# Autodesk Inventor assembly: Сборка1
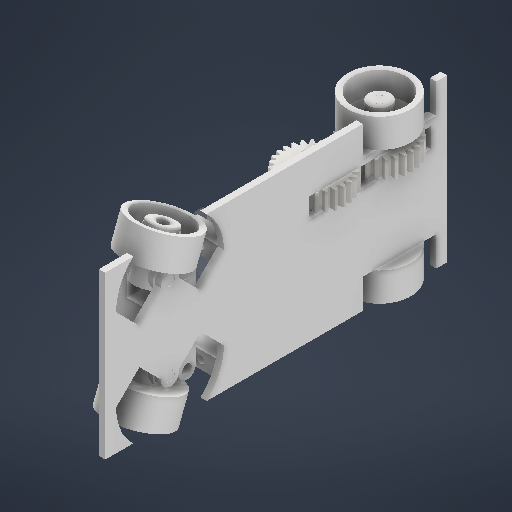
[picture p0: Inventor's stored thumbnail of the model, 512x512]
Saved by Autodesk Inventor 2026.2 (Build 302298000, 298)
## iProperties
Created: 2026-02-19
Part Number: Сборка1
Document SubType Name: Assembly
Designer: Leonid
Author: Leonid
## Documents named in this file (14)
- D:\Documents\Проекты\AutoBus\3Д модель\Сборка3.iam
- D:\Documents\Проекты\AutoBus\3Д модель\Малый сервопривод.ipt
- D:\Documents\Проекты\AutoBus\3Д модель\Рулевой толкатель на сервопривод.ipt
- D:\Documents\Проекты\AutoBus\3Д модель\Колесо переднее.ipt
- D:\Documents\Проекты\AutoBus\3Д модель\Кулак левый.ipt
- D:\Documents\Проекты\AutoBus\3Д модель\Штырь левый.ipt
- D:\Documents\Проекты\AutoBus\3Д модель\Тяга.ipt
- D:\Documents\Проекты\AutoBus\3Д модель\Кулак правый.ipt
- D:\Documents\Проекты\AutoBus\3Д модель\Штырь правый.ipt
- D:\Documents\Проекты\AutoBus\3Д модель\Вал.ipt
- D:\Documents\Проекты\AutoBus\3Д модель\Колесо заднее.ipt
- D:\Documents\Проекты\AutoBus\3Д модель\Рама3.ipt
- D:\Documents\Проекты\AutoBus\3Д модель\Мотор 15x12x10 с редуктоом.ipt
- D:\Documents\Проекты\AutoBus\3Д модель\Сборка3\Мастер проектирования\Цилиндрическое зубчатое зацепление4.iam
## Components (15 placed, 13 different names)
1. Рама3:1 — Цилиндрический:3, Совмещение:2, Заподлицо:2, Совмещение:12, Цилиндрический:16, Угол:1, Совмещение:13, Угол:2, Совмещение:19, Совмещение:20, Совмещение:24, Совмещение:25, Совмещение:26, Совмещение:28, Цилиндрический:26
2. Малый сервопривод:1 — Цилиндрический:11, Заподлицо:3, Совмещение:25, Совмещение:26
3. Кулак правый:1 — Цилиндрический:14, Совмещение:11, Совмещение:12, Цилиндрический:16, Цилиндрический:18, Заподлицо:7
4. Кулак левый:2 — Цилиндрический:3, Совмещение:2, Цилиндрический:4, Совмещение:4, Цилиндрический:13, Заподлицо:6
5. Тяга:1 — Цилиндрический:13, Цилиндрический:14, Совмещение:13, Касательность:1
6. Штырь правый:1 — Цилиндрический:17, Цилиндрический:18, Совмещение:14, Заподлицо:7
7. Штырь левый:2 — Цилиндрический:4, Цилиндрический:5, Совмещение:3, Заподлицо:6
8. Колесо переднее:1 — Совмещение:11, Цилиндрический:17, Совмещение:14
9. Колесо переднее:2 — Цилиндрический:5, Совмещение:3, Совмещение:4
10. Рулевой толкатель на сервопривод:1 — Цилиндрический:11, Заподлицо:3, Заподлицо:2, Угол:1, Угол:2, Касательность:1
11. Вал:1 — Цилиндрический:22, Заподлицо:8, Цилиндрический:23, Совмещение:27, Цилиндрический:25, Цилиндрический:26
12. Колесо заднее:1 — Цилиндрический:22, Совмещение:19, Заподлицо:8
13. Колесо заднее:2 — Цилиндрический:23, Совмещение:20
14. Мотор 15x12x10 с редуктоом:1 — Совмещение:24, Совмещение:27, Цилиндрический:24, Совмещение:29
15. Цилиндрическое зубчатое зацепление:2 [sub-assembly] — Цилиндрический:24, Цилиндрический:25, Совмещение:28, Совмещение:29
## Relationships (37: Mate 15, CylindricalJoint 14, Flush 5, Angle 2, Tangent 1)
- Цилиндрический:3 [CylindricalJoint]: Рама3:1 ↔ Кулак левый:2
- Совмещение:2 [Mate] (0.1 mm): Рама3:1 ↔ Кулак левый:2
- Заподлицо:2 [Flush] (-27.7 mm): Рама3:1 ↔ Рулевой толкатель на сервопривод:1
- Цилиндрический:4 [CylindricalJoint]: Кулак левый:2 ↔ Штырь левый:2
- Цилиндрический:5 [CylindricalJoint]: Штырь левый:2 ↔ Колесо переднее:2
- Совмещение:3 [Mate]: Штырь левый:2 ↔ Колесо переднее:2
- Совмещение:4 [Mate]: Кулак левый:2 ↔ Колесо переднее:2
- Цилиндрический:11 [CylindricalJoint]: Малый сервопривод:1 ↔ Рулевой толкатель на сервопривод:1
- Заподлицо:3 [Flush]: Малый сервопривод:1 ↔ Рулевой толкатель на сервопривод:1
- Цилиндрический:13 [CylindricalJoint]: Кулак левый:2 ↔ Тяга:1
- Цилиндрический:14 [CylindricalJoint]: Кулак правый:1 ↔ Тяга:1
- Совмещение:11 [Mate]: Кулак правый:1 ↔ Колесо переднее:1
- Совмещение:12 [Mate] (0.1 mm): Рама3:1 ↔ Кулак правый:1
- Цилиндрический:16 [CylindricalJoint]: Рама3:1 ↔ Кулак правый:1
- Угол:1 [Angle] (38 deg): Рама3:1 ↔ Рулевой толкатель на сервопривод:1
- Совмещение:13 [Mate] (0.15 mm): Рама3:1 ↔ Тяга:1
- Заподлицо:6 [Flush]: Кулак левый:2 ↔ Штырь левый:2
- Цилиндрический:17 [CylindricalJoint]: Штырь правый:1 ↔ Колесо переднее:1
- Цилиндрический:18 [CylindricalJoint]: Кулак правый:1 ↔ Штырь правый:1
- Совмещение:14 [Mate]: Штырь правый:1 ↔ Колесо переднее:1
- Заподлицо:7 [Flush]: Кулак правый:1 ↔ Штырь правый:1
- Угол:2 [Angle] (0 deg): Рама3:1 ↔ Рулевой толкатель на сервопривод:1
- Цилиндрический:22 [CylindricalJoint]: Вал:1 ↔ Колесо заднее:1
- Совмещение:19 [Mate] (0.25 mm): Рама3:1 ↔ Колесо заднее:1
- Заподлицо:8 [Flush]: Вал:1 ↔ Колесо заднее:1
- Цилиндрический:23 [CylindricalJoint]: Вал:1 ↔ Колесо заднее:2
- Совмещение:20 [Mate] (0.25 mm): Рама3:1 ↔ Колесо заднее:2
- Совмещение:24 [Mate]: Рама3:1 ↔ Мотор 15x12x10 с редуктоом:1
- Совмещение:25 [Mate]: Рама3:1 ↔ Малый сервопривод:1
- Совмещение:26 [Mate]: Рама3:1 ↔ Малый сервопривод:1
- Совмещение:27 [Mate] (17 mm): Вал:1 ↔ Мотор 15x12x10 с редуктоом:1
- Цилиндрический:24 [CylindricalJoint]: Мотор 15x12x10 с редуктоом:1 ↔ Цилиндрическое зубчатое зацепление:2
- Цилиндрический:25 [CylindricalJoint]: Вал:1 ↔ Цилиндрическое зубчатое зацепление:2
- Совмещение:28 [Mate] (0.15 mm): Рама3:1 ↔ Цилиндрическое зубчатое зацепление:2
- Касательность:1 [Tangent]: Тяга:1 ↔ Рулевой толкатель на сервопривод:1
- Цилиндрический:26 [CylindricalJoint]: Рама3:1 ↔ Вал:1
- Совмещение:29 [Mate]: Мотор 15x12x10 с редуктоом:1 ↔ Цилиндрическое зубчатое зацепление:2
